# Autodesk Inventor assembly: HbIndexFingerForChild
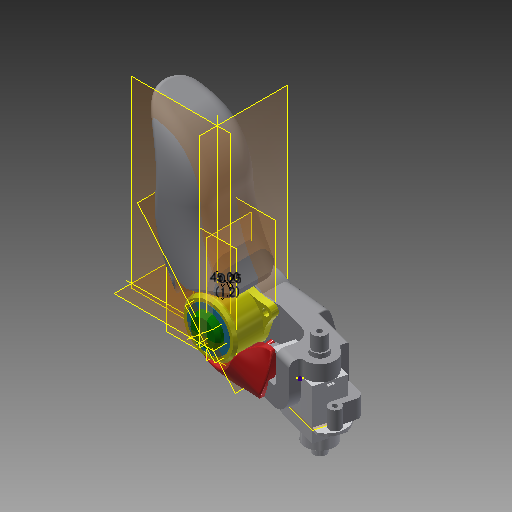
[picture p0: Inventor's stored thumbnail of the model, 512x512]
Saved by Autodesk Inventor 2017 (Build 210142000, 142)
## iProperties
Part Number: HbIndexFingerForChild
Material: 一般
Document SubType Name: Assembly
Designer: sktom
Author: sktom
## Documents named in this file (8)
- D:\OneDrive\CAD\MAJ\hackberry\HACKberry-hardware\3D_69%\Inventor\HbHandForChild\HbthumbU02ForChild\HbthumbU02ForChild.iam
- D:\OneDrive\CAD\MAJ\hackberry\HACKberry-hardware\3D_69%\Inventor\HbHandForChild\HbthumbU02ForChild\HbThumbMetacarpalPhalanx02ForChild.ipt
- D:\OneDrive\CAD\MAJ\hackberry\HACKberry-hardware\3D_69%\Inventor\HbHandForChild\HbthumbU02ForChild\HbThumbLockButton01ForChild.ipt
- D:\OneDrive\CAD\MAJ\hackberry\HACKberry-hardware\3D_69%\Inventor\HbHandForChild\HbthumbU02ForChild\HbThumbJointHolder01ForChild.ipt
- D:\OneDrive\CAD\MAJ\hackberry\HACKberry-hardware\3D_69%\Inventor\HbHandForChild\HbthumbU02ForChild\HbThumbProximalPhalanx02ForChild.ipt
- D:\OneDrive\CAD\MAJ\hackberry\HACKberry-hardware\3D_69%\Inventor\HbHandForChild\HbthumbU02ForChild\HbThumbProximalPhalanxBase02ForChild.ipt
- D:\OneDrive\CAD\MAJ\hackberry\HACKberry-hardware\3D_69%\Inventor\HbHandForChild\HbthumbU02ForChild\HbThumbMetacarpalPhalanxCover02ForChild.ipt
- D:\OneDrive\CAD\MAJ\hackberry\HACKberry-hardware\3D_69%\Inventor\HbHandForChild\HbthumbU02ForChild\HbServoHK282A\Servo_HK282A.ipt
## Components (7 placed, 7 different names)
1. HbThumbMetacarpalPhalanx02ForChild:1 — 挿入:1, 挿入:2, 挿入:3, 挿入:7, 挿入:8
2. HbThumbLockButton01ForChild:1 — 挿入:3
3. HbThumbJointHolder01ForChild:1 — 挿入:1, 挿入:2, 挿入:4, 挿入:6
4. HbThumbProximalPhalanx02ForChild:1 — 挿入:5
5. HbThumbProximalPhalanxBase02ForChild:1 — 挿入:4, 挿入:5
6. HbThumbMetacarpalPhalanxCover02ForChild:1 — 挿入:6
7. Servo_HK282A:1 — 挿入:7, 挿入:8
## Relationships (8: Insert 8)
- 挿入:1 [Insert]: HbThumbMetacarpalPhalanx02ForChild:1 ↔ HbThumbJointHolder01ForChild:1
- 挿入:2 [Insert]: HbThumbMetacarpalPhalanx02ForChild:1 ↔ HbThumbJointHolder01ForChild:1
- 挿入:3 [Insert] (2 mm): HbThumbMetacarpalPhalanx02ForChild:1 ↔ HbThumbLockButton01ForChild:1
- 挿入:4 [Insert]: HbThumbJointHolder01ForChild:1 ↔ HbThumbProximalPhalanxBase02ForChild:1
- 挿入:5 [Insert]: HbThumbProximalPhalanx02ForChild:1 ↔ HbThumbProximalPhalanxBase02ForChild:1
- 挿入:6 [Insert]: HbThumbJointHolder01ForChild:1 ↔ HbThumbMetacarpalPhalanxCover02ForChild:1
- 挿入:7 [Insert]: HbThumbMetacarpalPhalanx02ForChild:1 ↔ Servo_HK282A:1
- 挿入:8 [Insert]: HbThumbMetacarpalPhalanx02ForChild:1 ↔ Servo_HK282A:1
